# Autodesk Inventor assembly: chassisstructure
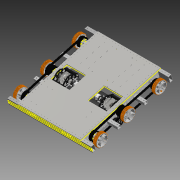
[picture p0: Inventor's stored thumbnail of the model, 180x180]
Saved by Autodesk Inventor 2014 SP1 (Build 180222100, 222)
## iProperties
Created: 2014-01-04
Part Number: chassisstructure
Document SubType Name: Assembly
Designer: Arpan
Mass: 20831.8 g
Surface Area: 51858.3 cm^2
Volume: 17520.2 cm^3
Density: 1.18902 g/cm^3
Author: Arpan
## Documents named in this file (29)
- C:\Users\Arpan\Documents\GitHub\2014buildCAD\chassisdrivetrain\chassis light\chassisstructure.iam
- C:\Users\Arpan\Documents\GitHub\2014buildCAD\chassisdrivetrain\chassis light\chassis side rail.ipt
- C:\Users\Arpan\Documents\GitHub\2014buildCAD\chassisdrivetrain\chassis light\COTS items\center wheel assembly.iam
- C:\Users\Arpan\Documents\GitHub\2014buildCAD\chassisdrivetrain\chassis light\COTS items\.5 inch bearing pretend its hex.ipt
- C:\Users\Arpan\Documents\GitHub\2014buildCAD\chassisdrivetrain\chassis light\4.5 hex shaft.ipt
- C:\Users\Arpan\Documents\GitHub\2014buildCAD\chassisdrivetrain\chassis light\COTS items\front wheels.iam
- C:\Users\Arpan\Documents\GitHub\2014buildCAD\chassisdrivetrain\chassis light\COTS items\back wheels.iam
- C:\Users\Arpan\Documents\GitHub\2014buildCAD\chassisdrivetrain\chassis light\COTS items\DBK_42ToothPulley V2.iam
- C:\Users\Arpan\Documents\GitHub\2014buildCAD\chassisdrivetrain\chassis light\3d printed items\back wheel spacer.ipt
- C:\Users\Arpan\Documents\GitHub\2014buildCAD\chassisdrivetrain\chassis light\PVC pipe spacer.ipt
- C:\Users\Arpan\Documents\GitHub\2014buildCAD\chassisdrivetrain\chassis light\PVC pipe spacer center wheels.ipt
- C:\Users\Arpan\Documents\GitHub\2014buildCAD\chassisdrivetrain\chassis light\baseplate.ipt
- C:\Users\Arpan\Documents\GitHub\2014buildCAD\chassisdrivetrain\chassis light\side bumper mount.ipt
- C:\Users\Arpan\Documents\GitHub\2014buildCAD\chassisdrivetrain\chassis light\COTS items\217-3547-STEP.ipt
- C:\Users\Arpan\Documents\GitHub\2014buildCAD\chassisdrivetrain\chassis light\front back rail vexpro.ipt
- C:\Users\Arpan\Documents\GitHub\2014buildCAD\chassisdrivetrain\chassis light\back rail vexpro.ipt
- C:\Users\Arpan\Documents\GitHub\2014buildCAD\chassisdrivetrain\chassis light\COTS items\HTD 5M-15 Belt 670mm.ipt
- C:\Users\Arpan\Documents\GitHub\2014buildCAD\chassisdrivetrain\chassis light\COTS items\HTD 5M-15 Belt 740mm.ipt
- C:\Users\Arpan\Documents\GitHub\2014buildCAD\chassisdrivetrain\chassis light\PVC pipe spacer front wheels.ipt
- C:\Users\Arpan\Documents\GitHub\2014buildCAD\Bumpers\Bumper Assembly2 (26x28 robot).iam
- C:\Users\Arpan\Documents\GitHub\2014buildCAD\Bumpers\Bumper Assembly3 (26x28 robot).iam
- C:\Users\Arpan\Documents\GitHub\2014buildCAD\Bumpers\Bumper Assembly4 (26x28 robot).iam
- C:\Users\Arpan\Documents\GitHub\2014buildCAD\chassisdrivetrain\gearbot\217-3433 (3 CIM Gearbox - WC)\217-3433-Fully Constrained.iam
- C:\Users\Arpan\Documents\GitHub\2014buildCAD\chassisdrivetrain\chassis light\battery staple.ipt
- C:\Users\Arpan\Documents\GitHub\2014buildCAD\chassisdrivetrain\chassis light\uderbodyweight.ipt
- C:\Users\Arpan\Documents\GitHub\2014buildCAD\Bumpers\Bumper Assembly1 (26x28 robot).iam
- C:\Users\Arpan\Documents\GitHub\2014buildCAD\hardware\10-24\thin hex locknut 90633A011.ipt
- C:\Users\Arpan\Documents\GitHub\2014buildCAD\chassisdrivetrain\chassis light\chassis hex hub clone.ipt
- C:\Users\Arpan\Documents\GitHub\2014buildCAD\chassisdrivetrain\chassis light\DXFs for steve\Part1.ipt
## Components (69 placed, 28 different names)
1. battery staple:1 — Mate:129, Mate:130, Mate:131
2. uderbodyweight:1 — Mate:132, Mate:133, Mate:134
3. thin hex locknut 90633A011:1 — Mate:149
4. thin hex locknut 90633A011:2 — Mate:152
5. thin hex locknut 90633A011:3 — Mate:156
6. thin hex locknut 90633A011:4 — Mate:158
7. thin hex locknut 90633A011:5 — Mate:150
8. thin hex locknut 90633A011:6 — Mate:154
9. chassis hex hub clone:1 — Mate:159, Mate:160, Mate:161, Mate:167, Mate:168, Mate:169, Mate:170, Mate:171, Mate:172
10. chassis hex hub clone:2 — Mate:164, Mate:165, Mate:166
11. thin hex locknut 90633A011:7 — Mate:167, Mate:177
12. thin hex locknut 90633A011:8 — Mate:168, Mate:173
13. thin hex locknut 90633A011:9 — Mate:170, Mate:175
14. thin hex locknut 90633A011:10 — Mate:172, Mate:174
15. thin hex locknut 90633A011:11 — Mate:169, Mate:178
16. thin hex locknut 90633A011:12 — Mate:171, Mate:176
17. Part1:1 — Flush:57
18. baseplate:1 — Flush:25, Mate:80, Mate:81, Flush:40, Mate:86, Mate:91, Flush:48, Mate:131, Mate:132, Mate:133, Mate:134
19. 217-3547-STEP:1 — Mate:75, Flush:31, Flush:32
20. 217-3547-STEP:2 — Mate:76, Flush:33, Flush:34
21. 217-3547-STEP:3 — Mate:77, Flush:35, Flush:36
22. 217-3547-STEP:4 — Mate:78, Flush:37, Flush:38
23. back rail vexpro:1 — Mate:91, Flush:47, Mate:92, Mate:125, Mate:126, Mate:129, Flush:54
24. front back rail vexpro:1 — Mate:80, Mate:81, Mate:82, Flush:39, Mate:83, Flush:40, Flush:41, Flush:44, Flush:46, Flush:47, Mate:124, Flush:49
25. chassis side rail:2 — Mate:21, Mate:22, Mate:23, Mate:24, Mate:25, Mate:26, Mate:27, Mate:28, Angle:3, Flush:25, Mate:70, Mate:71, Flush:26, Flush:27, Flush:36, Mate:78, Flush:37, Mate:82, Flush:39, Mate:86, Flush:43, Mate:97, Mate:98, Mate:103, Mate:104, Mate:130
26. chassis side rail:1 — Mate:14, Mate:15, Mate:16, Mate:17, Mate:18, Mate:19, Mate:20, Mate:29, Mate:72, Flush:28, Mate:73, Flush:29, Mate:75, Flush:31, Flush:33, Mate:83, Flush:41, Flush:43, Flush:44, Mate:92, Mate:94, Mate:95, Mate:100, Mate:101
27. side bumper mount:1 — Mate:70, Flush:27, Flush:30, Mate:77, Flush:35, Mate:90
28. side bumper mount:2 — Mate:71, Flush:26, Flush:38, Flush:45, Mate:90, Flush:46, Mate:137
29. side bumper mount:3 — Mate:72, Flush:28, Flush:30, Flush:32, Mate:135
30. side bumper mount:4 — Mate:73, Flush:29, Mate:76, Flush:34, Flush:45
31. PVC pipe spacer front wheels:1 — Mate:116, Mate:117
32. PVC pipe spacer center wheels:2 — Mate:112
33. PVC pipe spacer center wheels:1 — Mate:114
34. PVC pipe spacer front wheels:2 — Mate:118, Mate:119
35. PVC pipe spacer:1 — Mate:121
36. PVC pipe spacer:2 — Mate:123
37. HTD 5M-15 Belt 670mm:1 — Mate:100, Mate:101, Mate:102
38. HTD 5M-15 Belt 670mm:2 — Mate:103, Mate:104, Mate:105
39. HTD 5M-15 Belt 740mm:1 — Mate:94, Mate:95, Mate:96
40. HTD 5M-15 Belt 740mm:2 — Mate:97, Mate:98, Mate:99
41. 4.5 hex shaft:1 — Mate:30, Flush:9, Flush:13, Mate:36, Mate:37, Mate:119, Rotation:3
42. 4.5 hex shaft:2 — Mate:31, Flush:9, Flush:15, Mate:40, Mate:41, Mate:123, Rotation:4
43. 4.5 hex shaft:3 — Mate:32, Flush:11, Mate:34, Mate:35, Angle:3, Flush:19, Mate:117, Rotation:2
44. 4.5 hex shaft:4 — Flush:11, Mate:33, Mate:38, Mate:39, Flush:20, Mate:121, Flush:57
45. .5 inch bearing pretend its hex:1 — Mate:16, Mate:17
46. .5 inch bearing pretend its hex:2 — Mate:14, Mate:15, Mate:30
47. .5 inch bearing pretend its hex:3 — Mate:19, Mate:29
48. .5 inch bearing pretend its hex:4 — Mate:18, Mate:20, Mate:31
49. .5 inch bearing pretend its hex:5 — Mate:21, Mate:24, Mate:33
50. .5 inch bearing pretend its hex:6 — Mate:22, Mate:23
51. .5 inch bearing pretend its hex:7 — Mate:25, Mate:26, Mate:32
52. .5 inch bearing pretend its hex:8 — Mate:27, Mate:28
53. back wheel spacer:1 — Mate:47, Mate:48, Mate:49, Mate:145
54. back wheel spacer:2 — Mate:50, Mate:51, Mate:52, Mate:179
55. front wheels:1 [sub-assembly] — Mate:34, Mate:35, Flush:17, Flush:19, Mate:99, Mate:116
56. front wheels:2 [sub-assembly] — Flush:13, Mate:36, Mate:37, Flush:21, Mate:96, Mate:118
57. back wheels:1 [sub-assembly] — Flush:15, Mate:40, Mate:41, Mate:42, Mate:43, Mate:44, Mate:48, Mate:49, Mate:145, Mate:149, Mate:150, Mate:152, Mate:154, Mate:156, Mate:158, Mate:165, Mate:166
58. back wheels:2 [sub-assembly] — Mate:38, Mate:39, Mate:45, Mate:46, Flush:18, Flush:20, Mate:51, Mate:52, Rotation:1, Mate:160, Mate:161, Mate:162, Mate:163, Mate:173, Mate:174, Mate:175, Mate:176, Mate:177, Mate:178, Mate:179
59. DBK_42ToothPulley V2:1 [sub-assembly] — Mate:42, Mate:43, Mate:44, Flush:23, Mate:47, Mate:102, Mate:164
60. DBK_42ToothPulley V2:2 [sub-assembly] — Mate:45, Mate:46, Flush:22, Mate:50, Mate:105, Mate:159, Mate:162, Mate:163
61. 217-3433-Fully Constrained:1 [sub-assembly] — Rotation:3, Rotation:4
62. 217-3433-Fully Constrained:2 [sub-assembly] — Rotation:1, Rotation:2
63. center wheel assembly:1 [sub-assembly] — Flush:17, Flush:18, Flush:22, Mate:114
64. center wheel assembly:2 [sub-assembly] — Flush:21, Flush:23, Mate:112
65. Bumper Assembly1 (26x28 robot):2 [sub-assembly] — Mate:135, Mate:136, Flush:55
66. Bumper Assembly1 (26x28 robot):1 [sub-assembly] — Mate:137, Mate:138, Flush:56
67. Bumper Assembly2 (26x28 robot):1 [sub-assembly] — Mate:124, Flush:48, Flush:49, Flush:50, Flush:51, Flush:53, Mate:136, Flush:55, Mate:138
68. Bumper Assembly3 (26x28 robot):1 [sub-assembly] — Mate:126, Flush:50, Flush:53
69. Bumper Assembly4 (26x28 robot):1 [sub-assembly] — Mate:125, Flush:51, Flush:54, Flush:56
## Relationships (177: Mate 126, Flush 44, RelateRotation 4, Angle 3)
- [Mate]: chassis side rail:1 ↔ 217-3433-Fully Constrained:1
- [Mate]: chassis side rail:1 ↔ 217-3433-Fully Constrained:1
- [Mate]: chassis side rail:2 ↔ 217-3433-Fully Constrained:2
- [Mate]: chassis side rail:2 ↔ 217-3433-Fully Constrained:2
- [Angle] (0 deg): 217-3433-Fully Constrained:1 ↔ 217-3433-Fully Constrained:2
- [Flush]: 217-3433-Fully Constrained:2 ↔ center wheel assembly:1
- [Mate]: 217-3433-Fully Constrained:2 ↔ center wheel assembly:1
- [Mate]: 217-3433-Fully Constrained:2 ↔ center wheel assembly:1
- [Flush]: 217-3433-Fully Constrained:1 ↔ center wheel assembly:2
- [Mate]: 217-3433-Fully Constrained:1 ↔ center wheel assembly:2
- [Mate]: 217-3433-Fully Constrained:1 ↔ center wheel assembly:2
- Mate:14: chassis side rail:1 ↔ .5 inch bearing pretend its hex:2
- Mate:15: chassis side rail:1 ↔ .5 inch bearing pretend its hex:2
- Mate:16: chassis side rail:1 ↔ .5 inch bearing pretend its hex:1
- Mate:17: chassis side rail:1 ↔ .5 inch bearing pretend its hex:1
- Mate:18: chassis side rail:1 ↔ .5 inch bearing pretend its hex:4
- Mate:19: chassis side rail:1 ↔ .5 inch bearing pretend its hex:3
- Mate:20: chassis side rail:1 ↔ .5 inch bearing pretend its hex:4
- Mate:21: chassis side rail:2 ↔ .5 inch bearing pretend its hex:5
- Mate:22: chassis side rail:2 ↔ .5 inch bearing pretend its hex:6
- Mate:23: chassis side rail:2 ↔ .5 inch bearing pretend its hex:6
- Mate:24: chassis side rail:2 ↔ .5 inch bearing pretend its hex:5
- Mate:25: chassis side rail:2 ↔ .5 inch bearing pretend its hex:7
- Mate:26: chassis side rail:2 ↔ .5 inch bearing pretend its hex:7
- Mate:27: chassis side rail:2 ↔ .5 inch bearing pretend its hex:8
- Mate:28: chassis side rail:2 ↔ .5 inch bearing pretend its hex:8
- Mate:29: chassis side rail:1 ↔ .5 inch bearing pretend its hex:3
- Mate:30: 4.5 hex shaft:1 ↔ .5 inch bearing pretend its hex:2
- Mate:31: 4.5 hex shaft:2 ↔ .5 inch bearing pretend its hex:4
- Flush:9: 4.5 hex shaft:1 ↔ 4.5 hex shaft:2
- Mate:32: 4.5 hex shaft:3 ↔ .5 inch bearing pretend its hex:7
- Flush:11: 4.5 hex shaft:3 ↔ 4.5 hex shaft:4
- Mate:33: 4.5 hex shaft:4 ↔ .5 inch bearing pretend its hex:5
- Mate:34: 4.5 hex shaft:3 ↔ front wheels:1
- Mate:35: 4.5 hex shaft:3 ↔ front wheels:1
- Flush:13: 4.5 hex shaft:1 ↔ front wheels:2
- Mate:36: 4.5 hex shaft:1 ↔ front wheels:2
- Mate:37: 4.5 hex shaft:1 ↔ front wheels:2
- Mate:38: 4.5 hex shaft:4 ↔ back wheels:2
- Mate:39: 4.5 hex shaft:4 ↔ back wheels:2
- Flush:15: 4.5 hex shaft:2 ↔ back wheels:1
- Mate:40: 4.5 hex shaft:2 ↔ back wheels:1
- Mate:41: 4.5 hex shaft:2 ↔ back wheels:1
- Mate:42: back wheels:1 ↔ DBK_42ToothPulley V2:1
- Mate:43: back wheels:1 ↔ DBK_42ToothPulley V2:1
- Mate:44: back wheels:1 ↔ DBK_42ToothPulley V2:1
- Mate:45: back wheels:2 ↔ DBK_42ToothPulley V2:2
- Mate:46: back wheels:2 ↔ DBK_42ToothPulley V2:2
- Flush:17: front wheels:1 ↔ center wheel assembly:1
- Flush:18: back wheels:2 ↔ center wheel assembly:1
- Angle:3 (0 deg): chassis side rail:2 ↔ 4.5 hex shaft:3
- Flush:19: 4.5 hex shaft:3 ↔ front wheels:1
- Flush:20: 4.5 hex shaft:4 ↔ back wheels:2
- Flush:21: front wheels:2 ↔ center wheel assembly:2
- Flush:22: DBK_42ToothPulley V2:2 ↔ center wheel assembly:1
- Flush:23: DBK_42ToothPulley V2:1 ↔ center wheel assembly:2
- Mate:47: back wheel spacer:1 ↔ DBK_42ToothPulley V2:1
- Mate:48: back wheel spacer:1 ↔ back wheels:1
- Mate:49: back wheel spacer:1 ↔ back wheels:1
- Mate:50: back wheel spacer:2 ↔ DBK_42ToothPulley V2:2
- Mate:51: back wheel spacer:2 ↔ back wheels:2
- Mate:52: back wheel spacer:2 ↔ back wheels:2
- Flush:25: baseplate:1 ↔ chassis side rail:2
- Mate:70: chassis side rail:2 ↔ side bumper mount:1
- Mate:71: chassis side rail:2 ↔ side bumper mount:2
- Flush:26: chassis side rail:2 ↔ side bumper mount:2
- Flush:27: chassis side rail:2 ↔ side bumper mount:1
- Mate:72: chassis side rail:1 ↔ side bumper mount:3
- Flush:28: chassis side rail:1 ↔ side bumper mount:3
- Mate:73: chassis side rail:1 ↔ side bumper mount:4
- Flush:29: chassis side rail:1 ↔ side bumper mount:4
- Flush:30: side bumper mount:1 ↔ side bumper mount:3
- Mate:75: 217-3547-STEP:1 ↔ chassis side rail:1
- Flush:31: 217-3547-STEP:1 ↔ chassis side rail:1
- Flush:32: 217-3547-STEP:1 ↔ side bumper mount:3
- Mate:76: 217-3547-STEP:2 ↔ side bumper mount:4
- Flush:33: 217-3547-STEP:2 ↔ chassis side rail:1
- Flush:34: 217-3547-STEP:2 ↔ side bumper mount:4
- Mate:77: 217-3547-STEP:3 ↔ side bumper mount:1
- Flush:35: 217-3547-STEP:3 ↔ side bumper mount:1
- Flush:36: 217-3547-STEP:3 ↔ chassis side rail:2
- Mate:78: 217-3547-STEP:4 ↔ chassis side rail:2
- Flush:37: 217-3547-STEP:4 ↔ chassis side rail:2
- Flush:38: 217-3547-STEP:4 ↔ side bumper mount:2
- Mate:80: baseplate:1 ↔ front back rail vexpro:1
- Mate:81: baseplate:1 ↔ front back rail vexpro:1
- Mate:82: front back rail vexpro:1 ↔ chassis side rail:2
- Flush:39 (86.36 mm): front back rail vexpro:1 ↔ chassis side rail:2
- Mate:83: front back rail vexpro:1 ↔ chassis side rail:1
- Flush:40: baseplate:1 ↔ front back rail vexpro:1
- Flush:41: front back rail vexpro:1 ↔ chassis side rail:1
- Mate:86: baseplate:1 ↔ chassis side rail:2
- Flush:43: chassis side rail:2 ↔ chassis side rail:1
- Flush:44 (86.36 mm): front back rail vexpro:1 ↔ chassis side rail:1
- Flush:45: side bumper mount:2 ↔ side bumper mount:4
- Mate:90 (203.2 mm): side bumper mount:1 ↔ side bumper mount:2
- Flush:46 (-444.5 mm): front back rail vexpro:1 ↔ side bumper mount:2
- Mate:91: baseplate:1 ↔ back rail vexpro:1
- Flush:47: back rail vexpro:1 ↔ front back rail vexpro:1
- Mate:92: back rail vexpro:1 ↔ chassis side rail:1
- Mate:94: chassis side rail:1 ↔ HTD 5M-15 Belt 740mm:1
- Mate:95: chassis side rail:1 ↔ HTD 5M-15 Belt 740mm:1
- Mate:96 (0.7937 mm): HTD 5M-15 Belt 740mm:1 ↔ front wheels:2
- Mate:97: chassis side rail:2 ↔ HTD 5M-15 Belt 740mm:2
- Mate:98: chassis side rail:2 ↔ HTD 5M-15 Belt 740mm:2
- Mate:99 (0.7937 mm): HTD 5M-15 Belt 740mm:2 ↔ front wheels:1
- Mate:100: chassis side rail:1 ↔ HTD 5M-15 Belt 670mm:1
- Mate:101: chassis side rail:1 ↔ HTD 5M-15 Belt 670mm:1
- Mate:102 (0.7937 mm): HTD 5M-15 Belt 670mm:1 ↔ DBK_42ToothPulley V2:1
- Mate:103: chassis side rail:2 ↔ HTD 5M-15 Belt 670mm:2
- Mate:104: chassis side rail:2 ↔ HTD 5M-15 Belt 670mm:2
- Mate:105 (0.7937 mm): HTD 5M-15 Belt 670mm:2 ↔ DBK_42ToothPulley V2:2
- [Angle] (0 deg): back rail vexpro:1 ↔ 217-3433-Fully Constrained:2
- Mate:112: PVC pipe spacer center wheels:2 ↔ center wheel assembly:2
- [Mate]: PVC pipe spacer center wheels:2 ↔ 217-3433-Fully Constrained:1
- Mate:114: PVC pipe spacer center wheels:1 ↔ center wheel assembly:1
- [Mate]: PVC pipe spacer center wheels:1 ↔ 217-3433-Fully Constrained:2
- Mate:116: PVC pipe spacer front wheels:1 ↔ front wheels:1
- Mate:117: PVC pipe spacer front wheels:1 ↔ 4.5 hex shaft:3
- Mate:118: PVC pipe spacer front wheels:2 ↔ front wheels:2
- Mate:119: PVC pipe spacer front wheels:2 ↔ 4.5 hex shaft:1
- Mate:121: PVC pipe spacer:1 ↔ 4.5 hex shaft:4
- Mate:123: PVC pipe spacer:2 ↔ 4.5 hex shaft:2
- Mate:124: front back rail vexpro:1 ↔ Bumper Assembly2 (26x28 robot):1
- Flush:48 (25.4 mm): baseplate:1 ↔ Bumper Assembly2 (26x28 robot):1
- Flush:49 (-84.1375 mm): front back rail vexpro:1 ↔ Bumper Assembly2 (26x28 robot):1
- Mate:125: back rail vexpro:1 ↔ Bumper Assembly4 (26x28 robot):1
- Mate:126: back rail vexpro:1 ↔ Bumper Assembly3 (26x28 robot):1
- Flush:50: Bumper Assembly2 (26x28 robot):1 ↔ Bumper Assembly3 (26x28 robot):1
- Flush:51: Bumper Assembly2 (26x28 robot):1 ↔ Bumper Assembly4 (26x28 robot):1
- Flush:53: Bumper Assembly2 (26x28 robot):1 ↔ Bumper Assembly3 (26x28 robot):1
- Rotation:1 [RelateRotation] (1 ul): back wheels:2 ↔ 217-3433-Fully Constrained:2
- Rotation:2 [RelateRotation] (1 ul): 4.5 hex shaft:3 ↔ 217-3433-Fully Constrained:2
- Rotation:3 [RelateRotation] (1 ul): 4.5 hex shaft:1 ↔ 217-3433-Fully Constrained:1
- Rotation:4 [RelateRotation] (1 ul): 4.5 hex shaft:2 ↔ 217-3433-Fully Constrained:1
- Mate:129: battery staple:1 ↔ back rail vexpro:1
- Mate:130 (50.165 mm): battery staple:1 ↔ chassis side rail:2
- Mate:131: battery staple:1 ↔ baseplate:1
- Mate:132: uderbodyweight:1 ↔ baseplate:1
- Mate:133: uderbodyweight:1 ↔ baseplate:1
- Mate:134: uderbodyweight:1 ↔ baseplate:1
- Flush:54 (84.1375 mm): back rail vexpro:1 ↔ Bumper Assembly4 (26x28 robot):1
- Mate:135: side bumper mount:3 ↔ Bumper Assembly1 (26x28 robot):2
- Mate:136: Bumper Assembly1 (26x28 robot):2 ↔ Bumper Assembly2 (26x28 robot):1
- Flush:55: Bumper Assembly1 (26x28 robot):2 ↔ Bumper Assembly2 (26x28 robot):1
- Mate:137: side bumper mount:2 ↔ Bumper Assembly1 (26x28 robot):1
- Mate:138: Bumper Assembly1 (26x28 robot):1 ↔ Bumper Assembly2 (26x28 robot):1
- Flush:56: Bumper Assembly1 (26x28 robot):1 ↔ Bumper Assembly4 (26x28 robot):1
- Mate:145: back wheel spacer:1 ↔ back wheels:1
- Mate:149: thin hex locknut 90633A011:1 ↔ back wheels:1
- Mate:150: thin hex locknut 90633A011:5 ↔ back wheels:1
- Mate:152: thin hex locknut 90633A011:2 ↔ back wheels:1
- Mate:154: thin hex locknut 90633A011:6 ↔ back wheels:1
- Mate:156: thin hex locknut 90633A011:3 ↔ back wheels:1
- Mate:158: thin hex locknut 90633A011:4 ↔ back wheels:1
- Mate:159: chassis hex hub clone:1 ↔ DBK_42ToothPulley V2:2
- Mate:160: chassis hex hub clone:1 ↔ back wheels:2
- Mate:161: chassis hex hub clone:1 ↔ back wheels:2
- Mate:162: back wheels:2 ↔ DBK_42ToothPulley V2:2
- Mate:163: back wheels:2 ↔ DBK_42ToothPulley V2:2
- Mate:164: chassis hex hub clone:2 ↔ DBK_42ToothPulley V2:1
- Mate:165: chassis hex hub clone:2 ↔ back wheels:1
- Mate:166: chassis hex hub clone:2 ↔ back wheels:1
- Mate:167: chassis hex hub clone:1 ↔ thin hex locknut 90633A011:7
- Mate:168: chassis hex hub clone:1 ↔ thin hex locknut 90633A011:8
- Mate:169: chassis hex hub clone:1 ↔ thin hex locknut 90633A011:11
- Mate:170: chassis hex hub clone:1 ↔ thin hex locknut 90633A011:9
- Mate:171: chassis hex hub clone:1 ↔ thin hex locknut 90633A011:12
- Mate:172: chassis hex hub clone:1 ↔ thin hex locknut 90633A011:10
- Mate:173: thin hex locknut 90633A011:8 ↔ back wheels:2
- Mate:174: thin hex locknut 90633A011:10 ↔ back wheels:2
- Mate:175: thin hex locknut 90633A011:9 ↔ back wheels:2
- Mate:176: thin hex locknut 90633A011:12 ↔ back wheels:2
- Mate:177: thin hex locknut 90633A011:7 ↔ back wheels:2
- Mate:178: thin hex locknut 90633A011:11 ↔ back wheels:2
- Mate:179: back wheel spacer:2 ↔ back wheels:2
- Flush:57: Part1:1 ↔ 4.5 hex shaft:4
